# Autodesk Inventor assembly: リンク_6_1
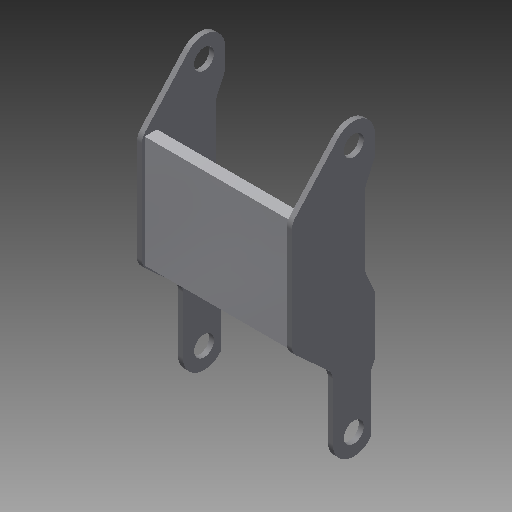
[picture p0: Inventor's stored thumbnail of the model, 512x512]
Saved by Autodesk Inventor 2018 (Build 220112000, 112)
## iProperties
Created: 2016-08-23
Part Number: リンク_6_1
Material: 一般
Document SubType Name: Assembly
Designer: hiro
Mass: 33.5175 g
Surface Area: 182.778 cm^2
Volume: 15.549 cm^3
Density: 2.15561 g/cm^3
Author: hiro
## Documents named in this file (3)
- Z:\OPR\OpenPlatform_ver1_0\下半身_160823\リンク\リンク_6_2.iam
- Z:\OPR\OpenPlatform_ver1_0\下半身_160823\リンク\リンク_メインフレーム_6_2.ipt
- Z:\OPR\OpenPlatform_ver1_0\下半身\リンク\ふくらはぎ\リンク_ふくらはぎ_サブフレーム_1_1(予備案).ipt
## Components (3 placed, 2 different names)
1. リンク_メインフレーム_6_2:1 — 挿入:17, 挿入:18, 挿入:19
2. リンク_メインフレーム_6_2:2 — 挿入:14, 挿入:15, 挿入:16
3. リンク_ふくらはぎ_サブフレーム_1_1(予備案):1 — 挿入:14, 挿入:15, 挿入:16, 挿入:17, 挿入:18, 挿入:19
## Relationships (6: Insert 6)
- 挿入:14 [Insert]: リンク_メインフレーム_6_2:2 ↔ リンク_ふくらはぎ_サブフレーム_1_1(予備案):1
- 挿入:15 [Insert]: リンク_メインフレーム_6_2:2 ↔ リンク_ふくらはぎ_サブフレーム_1_1(予備案):1
- 挿入:16 [Insert]: リンク_メインフレーム_6_2:2 ↔ リンク_ふくらはぎ_サブフレーム_1_1(予備案):1
- 挿入:17 [Insert]: リンク_メインフレーム_6_2:1 ↔ リンク_ふくらはぎ_サブフレーム_1_1(予備案):1
- 挿入:18 [Insert]: リンク_メインフレーム_6_2:1 ↔ リンク_ふくらはぎ_サブフレーム_1_1(予備案):1
- 挿入:19 [Insert]: リンク_メインフレーム_6_2:1 ↔ リンク_ふくらはぎ_サブフレーム_1_1(予備案):1
